# Autodesk Inventor assembly: StepperSystem
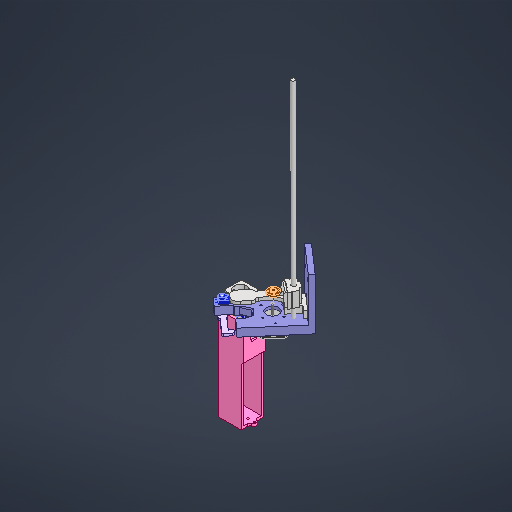
[picture p0: Inventor's stored thumbnail of the model, 512x512]
Saved by Autodesk Inventor 2025.1 (Build 291241000, 241)
## iProperties
Created: 2025-01-26
Part Number: StepperSystem
Document SubType Name: Assembly
Designer: 13156
Author: 13156
## Documents named in this file (12)
- C:\Users\jerem\Documents\GitHub\Perovskite-Automated-Synthesis-System\CAD\Pipette\StepperSystem.iam
- C:\Users\jerem\Documents\GitHub\Perovskite-Automated-Synthesis-System\CAD\Pipette\HolderWStepper.ipt
- C:\Users\jerem\Documents\GitHub\Perovskite-Automated-Synthesis-System\CAD\Non 3D Printed Parts\Linear Rails\8mm Linear Rod.ipt
- C:\Users\jerem\Documents\GitHub\Perovskite-Automated-Synthesis-System\CAD\Non 3D Printed Parts\Linear Rails\Linear Bearing 8mm Square.ipt
- C:\Users\jerem\Documents\GitHub\Perovskite-Automated-Synthesis-System\CAD\Pipette\Actuator.ipt
- C:\Users\jerem\Documents\GitHub\Perovskite-Automated-Synthesis-System\CAD\Pipette\PipetteStand.ipt
- C:\Users\jerem\Documents\GitHub\Perovskite-Automated-Synthesis-System\CAD\Non 3D Printed Parts\Motors and Servos\SG90 Servo.ipt
- C:\Users\jerem\Documents\GitHub\Perovskite-Automated-Synthesis-System\CAD\Pipette\GrabberArm.ipt
- C:\Users\jerem\Documents\GitHub\Perovskite-Automated-Synthesis-System\CAD\Pipette\SLEEVE.ipt
- C:\Users\jerem\Documents\GitHub\Perovskite-Automated-Synthesis-System\CAD\Non 3D Printed Parts\Leadscrew.ipt
- C:\Users\jerem\Documents\GitHub\Perovskite-Automated-Synthesis-System\CAD\Non 3D Printed Parts\Linear Rails\Linear Rod Holder SK8.ipt
- C:\Users\jerem\Documents\GitHub\Perovskite-Automated-Synthesis-System\CAD\Non 3D Printed Parts\Motors and Servos\NEMA17 Stepper Motor - 26 mm.ipt
## Components (14 placed, 11 different names)
1. HolderWStepper:1 — Mate:9, Mate:13, Mate:14, Mate:15, Mate:16, Mate:17, Mate:18, Mate:19, Mate:25, Mate:26, Mate:34, Mate:35, Mate:37, Flush:3, Mate:38, Mate:39, Mate:40, Flush:4
2. 8mm Linear Rod:1 — Mate:20, Mate:21, Flush:4
3. Linear Bearing 8mm Square:1 — Mate:21, Mate:28, Mate:29, Mate:30
4. Actuator:1 — Mate:28, Mate:29, Mate:30, Mate:31, Mate:32, Mate:33
5. PipetteStand:1 — Mate:1, Mate:2, Mate:3, Mate:4, Mate:5, Mate:6
6. SG90 Servo:1 — Mate:38, Mate:39, Mate:40, Mate:44
7. GrabberArm:1 — Mate:44
8. SLEEVE:1
9. Leadscrew:1 — Mate:31, Mate:32, Mate:33
10. Linear Rod Holder SK8:1 — Mate:13, Mate:14, Mate:15, Mate:16
11. Linear Rod Holder SK8:2 — Mate:17, Mate:18, Mate:19, Mate:20
12. SG90 Servo:3 — Mate:34, Mate:35
13. NEMA17 Stepper Motor - 26 mm:2 — Mate:9, Mate:25, Mate:26
14. SLEEVE:1 — Mate:4, Mate:5, Mate:6, Mate:37, Flush:3
## Relationships (33: Mate 31, Flush 2)
- Mate:1: PipetteStand:1
- Mate:2: PipetteStand:1
- Mate:3: PipetteStand:1
- Mate:4: PipetteStand:1 ↔ SLEEVE:1
- Mate:5 (0.75 mm): PipetteStand:1 ↔ SLEEVE:1
- Mate:6 (0.5 mm): PipetteStand:1 ↔ SLEEVE:1
- Mate:9: HolderWStepper:1 ↔ NEMA17 Stepper Motor - 26 mm:2
- Mate:13: HolderWStepper:1 ↔ Linear Rod Holder SK8:1
- Mate:14: HolderWStepper:1 ↔ Linear Rod Holder SK8:1
- Mate:15: HolderWStepper:1 ↔ Linear Rod Holder SK8:1
- Mate:16: HolderWStepper:1 ↔ Linear Rod Holder SK8:1
- Mate:17: HolderWStepper:1 ↔ Linear Rod Holder SK8:2
- Mate:18: HolderWStepper:1 ↔ Linear Rod Holder SK8:2
- Mate:19: HolderWStepper:1 ↔ Linear Rod Holder SK8:2
- Mate:20: 8mm Linear Rod:1 ↔ Linear Rod Holder SK8:2
- Mate:21: 8mm Linear Rod:1 ↔ Linear Bearing 8mm Square:1
- Mate:25: HolderWStepper:1 ↔ NEMA17 Stepper Motor - 26 mm:2
- Mate:26: HolderWStepper:1 ↔ NEMA17 Stepper Motor - 26 mm:2
- Mate:28: Linear Bearing 8mm Square:1 ↔ Actuator:1
- Mate:29: Linear Bearing 8mm Square:1 ↔ Actuator:1
- Mate:30: Linear Bearing 8mm Square:1 ↔ Actuator:1
- Mate:31: Actuator:1 ↔ Leadscrew:1
- Mate:32: Actuator:1 ↔ Leadscrew:1
- Mate:33: Actuator:1 ↔ Leadscrew:1
- Mate:34: HolderWStepper:1 ↔ SG90 Servo:3
- Mate:35: HolderWStepper:1 ↔ SG90 Servo:3
- Mate:37: HolderWStepper:1 ↔ SLEEVE:1
- Flush:3: HolderWStepper:1 ↔ SLEEVE:1
- Mate:38: HolderWStepper:1 ↔ SG90 Servo:1
- Mate:39: HolderWStepper:1 ↔ SG90 Servo:1
- Mate:40: HolderWStepper:1 ↔ SG90 Servo:1
- Mate:44: SG90 Servo:1 ↔ GrabberArm:1
- Flush:4: HolderWStepper:1 ↔ 8mm Linear Rod:1
